# Autodesk Inventor assembly: Stadio9
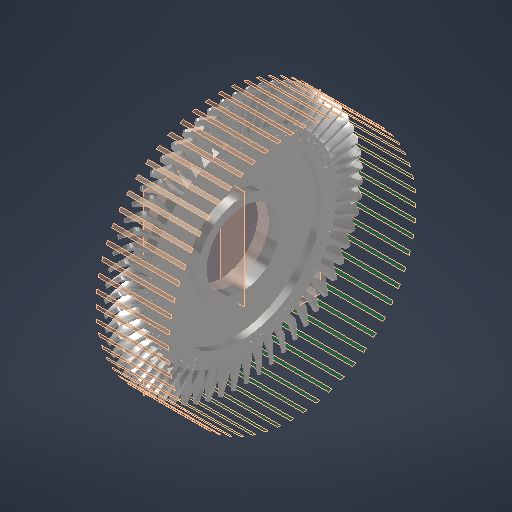
[picture p0: Inventor's stored thumbnail of the model, 512x512]
Saved by Autodesk Inventor 2026.2 (Build 302298010, 298A)
## iProperties
Created: 2026-04-25
Part Number: Stadio9
Document SubType Name: Assembly
Designer: Yan
Author: Yan
## Documents named in this file (3)
- C:\Users\Yan\Desktop\Turbina\Stadio9.iam
- C:\Users\Yan\Desktop\Turbina\DiscoPaleStadio9-DimensioniAprossimate.ipt
- C:\Users\Yan\Desktop\Turbina\PalaStadio9.ipt
## Components (61 placed, 2 different names)
1. DiscoPaleStadio9-DimensioniAprossimate:1 — Mate:1, Mate:2, Mate:3, Mate:4, Mate:5, Mate:6, Mate:7, Mate:8, Mate:9, Mate:10, Mate:11, Mate:12, Mate:13, Mate:14, Mate:15, Mate:16, Mate:17, Mate:18, Mate:19, Mate:20, Mate:21, Mate:22, Mate:23, Mate:24, Mate:25, Mate:26, Mate:27, Mate:28, Mate:30, Mate:32, Mate:33, Mate:34, Mate:35, Mate:36, Mate:37, Mate:38, Mate:39, Mate:40, Mate:41, Mate:42, Mate:43, Mate:44, Mate:45, Mate:46, Mate:47, Mate:48, Mate:49, Mate:50, Mate:51, Mate:52, Mate:53, Mate:54, Mate:55, Mate:56, Mate:57, Mate:58, Mate:59, Mate:60, Mate:61, Mate:62, Mate:63, Mate:64, Mate:65, Mate:66, Mate:67, Mate:68, Mate:69, Mate:70, Mate:71, Mate:72, Mate:73, Mate:74, Mate:75, Mate:76, Mate:77, Mate:78, Mate:79, Mate:80, Mate:81, Mate:82, Mate:83, Mate:84, Mate:85, Mate:86, Mate:87, Mate:88, Mate:89, Mate:90, Mate:91, Mate:92, Mate:93, Mate:94, Mate:95, Mate:96, Mate:97, Mate:98, Mate:99, Mate:100, Mate:101, Mate:102, Mate:103, Mate:104, Mate:105, Mate:106, Mate:107, Mate:108, Mate:109, Mate:110, Mate:111, Mate:112, Mate:113, Mate:114, Mate:115, Mate:116, Mate:117, Mate:118, Mate:119, Mate:120, Mate:121, Flush:1, Flush:2, Flush:3, Flush:4, Flush:5, Flush:6, Flush:7, Flush:8, Flush:9, Flush:10, Flush:11, Flush:12, Flush:13, Flush:14, Flush:15, Flush:16, Flush:17, Flush:18, Flush:19, Flush:20, Flush:21, Flush:22, Flush:23, Flush:24, Flush:25, Flush:26, Flush:27, Flush:28, Flush:29, Flush:30, Flush:31, Flush:32, Flush:33, Flush:34, Flush:35, Flush:36, Flush:37, Flush:38, Flush:39, Flush:40, Flush:41, Flush:42, Flush:43, Flush:44, Flush:45, Flush:46, Flush:47, Flush:48, Flush:49, Flush:50, Flush:51, Flush:52, Flush:53, Flush:54, Flush:55, Flush:56, Flush:57, Flush:58, Flush:59, Flush:60, Flush:61, Flush:62, Flush:63, Flush:64, Flush:65, Flush:66, Flush:67, Flush:68, Flush:69, Flush:70, Flush:71, Flush:72, Flush:73, Flush:74, Flush:75, Flush:76, Flush:77, Flush:78, Flush:79, Flush:80, Flush:81, Flush:82, Flush:83, Flush:84, Flush:85, Flush:86, Flush:87, Flush:88, Flush:89, Flush:90, Flush:91, Flush:92, Flush:93, Flush:94, Flush:95, Flush:96, Flush:97, Flush:98, Flush:99, Flush:100, Flush:101, Flush:102, Flush:103, Flush:104, Flush:105, Flush:106, Flush:107, Flush:108, Flush:109, Flush:110, Flush:111, Flush:112, Flush:113, Flush:114, Flush:115, Flush:116, Flush:117, Flush:118, Flush:119, Flush:120, Flush:121, Flush:122, Flush:123
2. PalaStadio9:1 — Mate:1, Mate:56, Flush:34, Flush:91
3. PalaStadio9:2 — Mate:2, Mate:55, Flush:33, Flush:90
4. PalaStadio9:3 — Mate:3, Mate:54, Flush:32, Flush:89
5. PalaStadio9:4 — Mate:4, Mate:58, Flush:31, Flush:88
6. PalaStadio9:5 — Mate:5, Mate:57, Flush:30, Flush:87
7. PalaStadio9:6 — Mate:6, Mate:53, Flush:29, Flush:86
8. PalaStadio9:7 — Mate:7, Mate:59, Flush:28, Flush:85
9. PalaStadio9:8 — Mate:8, Mate:52, Flush:27, Flush:84
10. PalaStadio9:9 — Mate:9, Mate:51, Flush:26, Flush:83
11. PalaStadio9:10 — Mate:10, Mate:50, Flush:25, Flush:82
12. PalaStadio9:11 — Mate:11, Mate:49, Flush:24, Flush:81
13. PalaStadio9:12 — Mate:12, Mate:42, Flush:23, Flush:80
14. PalaStadio9:13 — Mate:13, Mate:41, Flush:22, Flush:79
15. PalaStadio9:14 — Mate:14, Mate:48, Flush:21, Flush:78
16. PalaStadio9:15 — Mate:15, Mate:47, Flush:20, Flush:77
17. PalaStadio9:16 — Mate:16, Mate:46, Flush:19, Flush:76
18. PalaStadio9:17 — Mate:17, Mate:45, Flush:18, Flush:75
19. PalaStadio9:18 — Mate:18, Mate:40, Flush:17, Flush:74
20. PalaStadio9:19 — Mate:19, Mate:44, Flush:16, Flush:73
21. PalaStadio9:20 — Mate:20, Mate:43, Flush:15, Flush:72
22. PalaStadio9:21 — Mate:30, Mate:32, Flush:5, Flush:122
23. PalaStadio9:23 — Mate:28, Mate:60, Flush:7, Flush:61, Flush:62, Flush:64
24. PalaStadio9:24 — Mate:27, Mate:33, Flush:8, Flush:65
25. PalaStadio9:25 — Mate:26, Mate:34, Flush:9, Flush:66
26. PalaStadio9:26 — Mate:25, Mate:35, Flush:10, Flush:67
27. PalaStadio9:27 — Mate:24, Mate:36, Flush:11, Flush:68
28. PalaStadio9:28 — Mate:23, Mate:37, Flush:12, Flush:69
29. PalaStadio9:29 — Mate:22, Mate:38, Flush:13, Flush:70
30. PalaStadio9:30 — Mate:21, Mate:39, Flush:14, Flush:71
31. PalaStadio9:31 — Mate:62, Mate:65, Flush:36, Flush:93
32. PalaStadio9:32 — Mate:63, Mate:66, Flush:37, Flush:94
33. PalaStadio9:33 — Mate:67, Mate:68, Flush:38, Flush:95
34. PalaStadio9:34 — Mate:69, Mate:109, Flush:39, Flush:96
35. PalaStadio9:35 — Mate:70, Mate:110, Flush:40, Flush:97
36. PalaStadio9:36 — Mate:71, Mate:111, Flush:41, Flush:98
37. PalaStadio9:37 — Mate:72, Mate:112, Flush:42, Flush:99
38. PalaStadio9:38 — Mate:73, Mate:113, Flush:43, Flush:100
39. PalaStadio9:39 — Mate:74, Mate:114, Flush:44, Flush:101
40. PalaStadio9:40 — Mate:61, Mate:64, Flush:35, Flush:92
41. PalaStadio9:41 — Mate:75, Mate:115, Flush:45, Flush:102
42. PalaStadio9:42 — Mate:76, Mate:116, Flush:46, Flush:103
43. PalaStadio9:43 — Mate:77, Mate:117, Flush:47, Flush:104
44. PalaStadio9:44 — Mate:78, Mate:118, Flush:48, Flush:105
45. PalaStadio9:45 — Mate:79, Mate:119, Flush:49, Flush:106
46. PalaStadio9:46 — Mate:80, Flush:50, Flush:107
47. PalaStadio9:47 — Mate:81, Mate:108, Flush:51, Flush:108
48. PalaStadio9:48 — Mate:82, Mate:107, Flush:52, Flush:109
49. PalaStadio9:49 — Mate:83, Mate:106, Flush:53, Flush:110
50. PalaStadio9:50 — Mate:84, Mate:105, Flush:54, Flush:111
51. PalaStadio9:51 — Mate:85, Mate:104, Flush:55, Flush:112
52. PalaStadio9:52 — Mate:86, Mate:103, Flush:56, Flush:113
53. PalaStadio9:53 — Mate:87, Mate:102, Flush:57, Flush:114
54. PalaStadio9:54 — Mate:88, Mate:101, Flush:58, Flush:115
55. PalaStadio9:55 — Mate:89, Mate:100, Flush:59, Flush:116
56. PalaStadio9:56 — Mate:90, Mate:99, Flush:60, Flush:117
57. PalaStadio9:57 — Mate:91, Mate:98, Flush:1, Flush:118
58. PalaStadio9:58 — Mate:92, Mate:97, Flush:2, Flush:119
59. PalaStadio9:59 — Mate:93, Mate:96, Flush:3, Flush:120
60. PalaStadio9:60 — Mate:94, Mate:95, Flush:6, Flush:63, Flush:123
61. PalaStadio9:61 — Mate:120, Mate:121, Flush:4, Flush:121
## Relationships (242: Flush 123, Mate 119)
- Mate:1: DiscoPaleStadio9-DimensioniAprossimate:1 ↔ PalaStadio9:1
- Mate:2: DiscoPaleStadio9-DimensioniAprossimate:1 ↔ PalaStadio9:2
- Mate:3: DiscoPaleStadio9-DimensioniAprossimate:1 ↔ PalaStadio9:3
- Mate:4: DiscoPaleStadio9-DimensioniAprossimate:1 ↔ PalaStadio9:4
- Mate:5: DiscoPaleStadio9-DimensioniAprossimate:1 ↔ PalaStadio9:5
- Mate:6: DiscoPaleStadio9-DimensioniAprossimate:1 ↔ PalaStadio9:6
- Mate:7: DiscoPaleStadio9-DimensioniAprossimate:1 ↔ PalaStadio9:7
- Mate:8: DiscoPaleStadio9-DimensioniAprossimate:1 ↔ PalaStadio9:8
- Mate:9: DiscoPaleStadio9-DimensioniAprossimate:1 ↔ PalaStadio9:9
- Mate:10: DiscoPaleStadio9-DimensioniAprossimate:1 ↔ PalaStadio9:10
- Mate:11: DiscoPaleStadio9-DimensioniAprossimate:1 ↔ PalaStadio9:11
- Mate:12: DiscoPaleStadio9-DimensioniAprossimate:1 ↔ PalaStadio9:12
- Mate:13: DiscoPaleStadio9-DimensioniAprossimate:1 ↔ PalaStadio9:13
- Mate:14: DiscoPaleStadio9-DimensioniAprossimate:1 ↔ PalaStadio9:14
- Mate:15: DiscoPaleStadio9-DimensioniAprossimate:1 ↔ PalaStadio9:15
- Mate:16: DiscoPaleStadio9-DimensioniAprossimate:1 ↔ PalaStadio9:16
- Mate:17: DiscoPaleStadio9-DimensioniAprossimate:1 ↔ PalaStadio9:17
- Mate:18: DiscoPaleStadio9-DimensioniAprossimate:1 ↔ PalaStadio9:18
- Mate:19: DiscoPaleStadio9-DimensioniAprossimate:1 ↔ PalaStadio9:19
- Mate:20: DiscoPaleStadio9-DimensioniAprossimate:1 ↔ PalaStadio9:20
- Mate:21: DiscoPaleStadio9-DimensioniAprossimate:1 ↔ PalaStadio9:30
- Mate:22: DiscoPaleStadio9-DimensioniAprossimate:1 ↔ PalaStadio9:29
- Mate:23: DiscoPaleStadio9-DimensioniAprossimate:1 ↔ PalaStadio9:28
- Mate:24: DiscoPaleStadio9-DimensioniAprossimate:1 ↔ PalaStadio9:27
- Mate:25: DiscoPaleStadio9-DimensioniAprossimate:1 ↔ PalaStadio9:26
- Mate:26: DiscoPaleStadio9-DimensioniAprossimate:1 ↔ PalaStadio9:25
- Mate:27: DiscoPaleStadio9-DimensioniAprossimate:1 ↔ PalaStadio9:24
- Mate:28: DiscoPaleStadio9-DimensioniAprossimate:1 ↔ PalaStadio9:23
- Mate:30: DiscoPaleStadio9-DimensioniAprossimate:1 ↔ PalaStadio9:21
- Mate:32: DiscoPaleStadio9-DimensioniAprossimate:1 ↔ PalaStadio9:21
- Mate:33: DiscoPaleStadio9-DimensioniAprossimate:1 ↔ PalaStadio9:24
- Mate:34: DiscoPaleStadio9-DimensioniAprossimate:1 ↔ PalaStadio9:25
- Mate:35: DiscoPaleStadio9-DimensioniAprossimate:1 ↔ PalaStadio9:26
- Mate:36: DiscoPaleStadio9-DimensioniAprossimate:1 ↔ PalaStadio9:27
- Mate:37: DiscoPaleStadio9-DimensioniAprossimate:1 ↔ PalaStadio9:28
- Mate:38: DiscoPaleStadio9-DimensioniAprossimate:1 ↔ PalaStadio9:29
- Mate:39: DiscoPaleStadio9-DimensioniAprossimate:1 ↔ PalaStadio9:30
- Mate:40: DiscoPaleStadio9-DimensioniAprossimate:1 ↔ PalaStadio9:18
- Mate:41: DiscoPaleStadio9-DimensioniAprossimate:1 ↔ PalaStadio9:13
- Mate:42: DiscoPaleStadio9-DimensioniAprossimate:1 ↔ PalaStadio9:12
- Mate:43: DiscoPaleStadio9-DimensioniAprossimate:1 ↔ PalaStadio9:20
- Mate:44: DiscoPaleStadio9-DimensioniAprossimate:1 ↔ PalaStadio9:19
- Mate:45: DiscoPaleStadio9-DimensioniAprossimate:1 ↔ PalaStadio9:17
- Mate:46: DiscoPaleStadio9-DimensioniAprossimate:1 ↔ PalaStadio9:16
- Mate:47: DiscoPaleStadio9-DimensioniAprossimate:1 ↔ PalaStadio9:15
- Mate:48: DiscoPaleStadio9-DimensioniAprossimate:1 ↔ PalaStadio9:14
- Mate:49: DiscoPaleStadio9-DimensioniAprossimate:1 ↔ PalaStadio9:11
- Mate:50: DiscoPaleStadio9-DimensioniAprossimate:1 ↔ PalaStadio9:10
- Mate:51: DiscoPaleStadio9-DimensioniAprossimate:1 ↔ PalaStadio9:9
- Mate:52: DiscoPaleStadio9-DimensioniAprossimate:1 ↔ PalaStadio9:8
- Mate:53: DiscoPaleStadio9-DimensioniAprossimate:1 ↔ PalaStadio9:6
- Mate:54: DiscoPaleStadio9-DimensioniAprossimate:1 ↔ PalaStadio9:3
- Mate:55: DiscoPaleStadio9-DimensioniAprossimate:1 ↔ PalaStadio9:2
- Mate:56: DiscoPaleStadio9-DimensioniAprossimate:1 ↔ PalaStadio9:1
- Mate:57: DiscoPaleStadio9-DimensioniAprossimate:1 ↔ PalaStadio9:5
- Mate:58: DiscoPaleStadio9-DimensioniAprossimate:1 ↔ PalaStadio9:4
- Mate:59: DiscoPaleStadio9-DimensioniAprossimate:1 ↔ PalaStadio9:7
- Mate:60: DiscoPaleStadio9-DimensioniAprossimate:1 ↔ PalaStadio9:23
- Mate:61: DiscoPaleStadio9-DimensioniAprossimate:1 ↔ PalaStadio9:40
- Mate:62: DiscoPaleStadio9-DimensioniAprossimate:1 ↔ PalaStadio9:31
- Mate:63: DiscoPaleStadio9-DimensioniAprossimate:1 ↔ PalaStadio9:32
- Mate:64: DiscoPaleStadio9-DimensioniAprossimate:1 ↔ PalaStadio9:40
- Mate:65: DiscoPaleStadio9-DimensioniAprossimate:1 ↔ PalaStadio9:31
- Mate:66: DiscoPaleStadio9-DimensioniAprossimate:1 ↔ PalaStadio9:32
- Mate:67: DiscoPaleStadio9-DimensioniAprossimate:1 ↔ PalaStadio9:33
- Mate:68: DiscoPaleStadio9-DimensioniAprossimate:1 ↔ PalaStadio9:33
- Mate:69: DiscoPaleStadio9-DimensioniAprossimate:1 ↔ PalaStadio9:34
- Mate:70: DiscoPaleStadio9-DimensioniAprossimate:1 ↔ PalaStadio9:35
- Mate:71: DiscoPaleStadio9-DimensioniAprossimate:1 ↔ PalaStadio9:36
- Mate:72: DiscoPaleStadio9-DimensioniAprossimate:1 ↔ PalaStadio9:37
- Mate:73: DiscoPaleStadio9-DimensioniAprossimate:1 ↔ PalaStadio9:38
- Mate:74: DiscoPaleStadio9-DimensioniAprossimate:1 ↔ PalaStadio9:39
- Mate:75: DiscoPaleStadio9-DimensioniAprossimate:1 ↔ PalaStadio9:41
- Mate:76: DiscoPaleStadio9-DimensioniAprossimate:1 ↔ PalaStadio9:42
- Mate:77: DiscoPaleStadio9-DimensioniAprossimate:1 ↔ PalaStadio9:43
- Mate:78: DiscoPaleStadio9-DimensioniAprossimate:1 ↔ PalaStadio9:44
- Mate:79: DiscoPaleStadio9-DimensioniAprossimate:1 ↔ PalaStadio9:45
- Mate:80: DiscoPaleStadio9-DimensioniAprossimate:1 ↔ PalaStadio9:46
- Mate:81: DiscoPaleStadio9-DimensioniAprossimate:1 ↔ PalaStadio9:47
- Mate:82: DiscoPaleStadio9-DimensioniAprossimate:1 ↔ PalaStadio9:48
- Mate:83: DiscoPaleStadio9-DimensioniAprossimate:1 ↔ PalaStadio9:49
- Mate:84: DiscoPaleStadio9-DimensioniAprossimate:1 ↔ PalaStadio9:50
- Mate:85: DiscoPaleStadio9-DimensioniAprossimate:1 ↔ PalaStadio9:51
- Mate:86: DiscoPaleStadio9-DimensioniAprossimate:1 ↔ PalaStadio9:52
- Mate:87: DiscoPaleStadio9-DimensioniAprossimate:1 ↔ PalaStadio9:53
- Mate:88: DiscoPaleStadio9-DimensioniAprossimate:1 ↔ PalaStadio9:54
- Mate:89: DiscoPaleStadio9-DimensioniAprossimate:1 ↔ PalaStadio9:55
- Mate:90: DiscoPaleStadio9-DimensioniAprossimate:1 ↔ PalaStadio9:56
- Mate:91: DiscoPaleStadio9-DimensioniAprossimate:1 ↔ PalaStadio9:57
- Mate:92: DiscoPaleStadio9-DimensioniAprossimate:1 ↔ PalaStadio9:58
- Mate:93: DiscoPaleStadio9-DimensioniAprossimate:1 ↔ PalaStadio9:59
- Mate:94: DiscoPaleStadio9-DimensioniAprossimate:1 ↔ PalaStadio9:60
- Mate:95: DiscoPaleStadio9-DimensioniAprossimate:1 ↔ PalaStadio9:60
- Mate:96: DiscoPaleStadio9-DimensioniAprossimate:1 ↔ PalaStadio9:59
- Mate:97: DiscoPaleStadio9-DimensioniAprossimate:1 ↔ PalaStadio9:58
- Mate:98: DiscoPaleStadio9-DimensioniAprossimate:1 ↔ PalaStadio9:57
- Mate:99: DiscoPaleStadio9-DimensioniAprossimate:1 ↔ PalaStadio9:56
- Mate:100: DiscoPaleStadio9-DimensioniAprossimate:1 ↔ PalaStadio9:55
- Mate:101: DiscoPaleStadio9-DimensioniAprossimate:1 ↔ PalaStadio9:54
- Mate:102: DiscoPaleStadio9-DimensioniAprossimate:1 ↔ PalaStadio9:53
- Mate:103: DiscoPaleStadio9-DimensioniAprossimate:1 ↔ PalaStadio9:52
- Mate:104: DiscoPaleStadio9-DimensioniAprossimate:1 ↔ PalaStadio9:51
- Mate:105: DiscoPaleStadio9-DimensioniAprossimate:1 ↔ PalaStadio9:50
- Mate:106: DiscoPaleStadio9-DimensioniAprossimate:1 ↔ PalaStadio9:49
- Mate:107: DiscoPaleStadio9-DimensioniAprossimate:1 ↔ PalaStadio9:48
- Mate:108: DiscoPaleStadio9-DimensioniAprossimate:1 ↔ PalaStadio9:47
- Mate:109: DiscoPaleStadio9-DimensioniAprossimate:1 ↔ PalaStadio9:34
- Mate:110: DiscoPaleStadio9-DimensioniAprossimate:1 ↔ PalaStadio9:35
- Mate:111: DiscoPaleStadio9-DimensioniAprossimate:1 ↔ PalaStadio9:36
- Mate:112: DiscoPaleStadio9-DimensioniAprossimate:1 ↔ PalaStadio9:37
- Mate:113: DiscoPaleStadio9-DimensioniAprossimate:1 ↔ PalaStadio9:38
- Mate:114: DiscoPaleStadio9-DimensioniAprossimate:1 ↔ PalaStadio9:39
- Mate:115: DiscoPaleStadio9-DimensioniAprossimate:1 ↔ PalaStadio9:41
- Mate:116: DiscoPaleStadio9-DimensioniAprossimate:1 ↔ PalaStadio9:42
- Mate:117: DiscoPaleStadio9-DimensioniAprossimate:1 ↔ PalaStadio9:43
- Mate:118: DiscoPaleStadio9-DimensioniAprossimate:1 ↔ PalaStadio9:44
- Mate:119: DiscoPaleStadio9-DimensioniAprossimate:1 ↔ PalaStadio9:45
- Mate:120: DiscoPaleStadio9-DimensioniAprossimate:1 ↔ PalaStadio9:61
- Mate:121: DiscoPaleStadio9-DimensioniAprossimate:1 ↔ PalaStadio9:61
- Flush:1: DiscoPaleStadio9-DimensioniAprossimate:1 ↔ PalaStadio9:57
- Flush:2: DiscoPaleStadio9-DimensioniAprossimate:1 ↔ PalaStadio9:58
- Flush:3: DiscoPaleStadio9-DimensioniAprossimate:1 ↔ PalaStadio9:59
- Flush:4: DiscoPaleStadio9-DimensioniAprossimate:1 ↔ PalaStadio9:61
- Flush:5: DiscoPaleStadio9-DimensioniAprossimate:1 ↔ PalaStadio9:21
- Flush:6: DiscoPaleStadio9-DimensioniAprossimate:1 ↔ PalaStadio9:60
- Flush:7: DiscoPaleStadio9-DimensioniAprossimate:1 ↔ PalaStadio9:23
- Flush:8: DiscoPaleStadio9-DimensioniAprossimate:1 ↔ PalaStadio9:24
- Flush:9: DiscoPaleStadio9-DimensioniAprossimate:1 ↔ PalaStadio9:25
- Flush:10: DiscoPaleStadio9-DimensioniAprossimate:1 ↔ PalaStadio9:26
- Flush:11: DiscoPaleStadio9-DimensioniAprossimate:1 ↔ PalaStadio9:27
- Flush:12: DiscoPaleStadio9-DimensioniAprossimate:1 ↔ PalaStadio9:28
- Flush:13: DiscoPaleStadio9-DimensioniAprossimate:1 ↔ PalaStadio9:29
- Flush:14: DiscoPaleStadio9-DimensioniAprossimate:1 ↔ PalaStadio9:30
- Flush:15: DiscoPaleStadio9-DimensioniAprossimate:1 ↔ PalaStadio9:20
- Flush:16: DiscoPaleStadio9-DimensioniAprossimate:1 ↔ PalaStadio9:19
- Flush:17: DiscoPaleStadio9-DimensioniAprossimate:1 ↔ PalaStadio9:18
- Flush:18: DiscoPaleStadio9-DimensioniAprossimate:1 ↔ PalaStadio9:17
- Flush:19: DiscoPaleStadio9-DimensioniAprossimate:1 ↔ PalaStadio9:16
- Flush:20: DiscoPaleStadio9-DimensioniAprossimate:1 ↔ PalaStadio9:15
- Flush:21: DiscoPaleStadio9-DimensioniAprossimate:1 ↔ PalaStadio9:14
- Flush:22: DiscoPaleStadio9-DimensioniAprossimate:1 ↔ PalaStadio9:13
- Flush:23: DiscoPaleStadio9-DimensioniAprossimate:1 ↔ PalaStadio9:12
- Flush:24: DiscoPaleStadio9-DimensioniAprossimate:1 ↔ PalaStadio9:11
- Flush:25: DiscoPaleStadio9-DimensioniAprossimate:1 ↔ PalaStadio9:10
- Flush:26: DiscoPaleStadio9-DimensioniAprossimate:1 ↔ PalaStadio9:9
- Flush:27: DiscoPaleStadio9-DimensioniAprossimate:1 ↔ PalaStadio9:8
- Flush:28: DiscoPaleStadio9-DimensioniAprossimate:1 ↔ PalaStadio9:7
- Flush:29: DiscoPaleStadio9-DimensioniAprossimate:1 ↔ PalaStadio9:6
- Flush:30: DiscoPaleStadio9-DimensioniAprossimate:1 ↔ PalaStadio9:5
- Flush:31: DiscoPaleStadio9-DimensioniAprossimate:1 ↔ PalaStadio9:4
- Flush:32: DiscoPaleStadio9-DimensioniAprossimate:1 ↔ PalaStadio9:3
- Flush:33: DiscoPaleStadio9-DimensioniAprossimate:1 ↔ PalaStadio9:2
- Flush:34: DiscoPaleStadio9-DimensioniAprossimate:1 ↔ PalaStadio9:1
- Flush:35: DiscoPaleStadio9-DimensioniAprossimate:1 ↔ PalaStadio9:40
- Flush:36: DiscoPaleStadio9-DimensioniAprossimate:1 ↔ PalaStadio9:31
- Flush:37: DiscoPaleStadio9-DimensioniAprossimate:1 ↔ PalaStadio9:32
- Flush:38: DiscoPaleStadio9-DimensioniAprossimate:1 ↔ PalaStadio9:33
- Flush:39: DiscoPaleStadio9-DimensioniAprossimate:1 ↔ PalaStadio9:34
- Flush:40: DiscoPaleStadio9-DimensioniAprossimate:1 ↔ PalaStadio9:35
- Flush:41: DiscoPaleStadio9-DimensioniAprossimate:1 ↔ PalaStadio9:36
- Flush:42: DiscoPaleStadio9-DimensioniAprossimate:1 ↔ PalaStadio9:37
- Flush:43: DiscoPaleStadio9-DimensioniAprossimate:1 ↔ PalaStadio9:38
- Flush:44: DiscoPaleStadio9-DimensioniAprossimate:1 ↔ PalaStadio9:39
- Flush:45: DiscoPaleStadio9-DimensioniAprossimate:1 ↔ PalaStadio9:41
- Flush:46: DiscoPaleStadio9-DimensioniAprossimate:1 ↔ PalaStadio9:42
- Flush:47: DiscoPaleStadio9-DimensioniAprossimate:1 ↔ PalaStadio9:43
- Flush:48: DiscoPaleStadio9-DimensioniAprossimate:1 ↔ PalaStadio9:44
- Flush:49: DiscoPaleStadio9-DimensioniAprossimate:1 ↔ PalaStadio9:45
- Flush:50: DiscoPaleStadio9-DimensioniAprossimate:1 ↔ PalaStadio9:46
- Flush:51: DiscoPaleStadio9-DimensioniAprossimate:1 ↔ PalaStadio9:47
- Flush:52: DiscoPaleStadio9-DimensioniAprossimate:1 ↔ PalaStadio9:48
- Flush:53: DiscoPaleStadio9-DimensioniAprossimate:1 ↔ PalaStadio9:49
- Flush:54: DiscoPaleStadio9-DimensioniAprossimate:1 ↔ PalaStadio9:50
- Flush:55: DiscoPaleStadio9-DimensioniAprossimate:1 ↔ PalaStadio9:51
- Flush:56: DiscoPaleStadio9-DimensioniAprossimate:1 ↔ PalaStadio9:52
- Flush:57: DiscoPaleStadio9-DimensioniAprossimate:1 ↔ PalaStadio9:53
- Flush:58: DiscoPaleStadio9-DimensioniAprossimate:1 ↔ PalaStadio9:54
- Flush:59: DiscoPaleStadio9-DimensioniAprossimate:1 ↔ PalaStadio9:55
- Flush:60: DiscoPaleStadio9-DimensioniAprossimate:1 ↔ PalaStadio9:56
- Flush:61: DiscoPaleStadio9-DimensioniAprossimate:1 ↔ PalaStadio9:23
- Flush:62: DiscoPaleStadio9-DimensioniAprossimate:1 ↔ PalaStadio9:23
- Flush:63: DiscoPaleStadio9-DimensioniAprossimate:1 ↔ PalaStadio9:60
- Flush:64: DiscoPaleStadio9-DimensioniAprossimate:1 ↔ PalaStadio9:23
- Flush:65: DiscoPaleStadio9-DimensioniAprossimate:1 ↔ PalaStadio9:24
- Flush:66: DiscoPaleStadio9-DimensioniAprossimate:1 ↔ PalaStadio9:25
- Flush:67: DiscoPaleStadio9-DimensioniAprossimate:1 ↔ PalaStadio9:26
- Flush:68: DiscoPaleStadio9-DimensioniAprossimate:1 ↔ PalaStadio9:27
- Flush:69: DiscoPaleStadio9-DimensioniAprossimate:1 ↔ PalaStadio9:28
- Flush:70: DiscoPaleStadio9-DimensioniAprossimate:1 ↔ PalaStadio9:29
- Flush:71: DiscoPaleStadio9-DimensioniAprossimate:1 ↔ PalaStadio9:30
- Flush:72: DiscoPaleStadio9-DimensioniAprossimate:1 ↔ PalaStadio9:20
- Flush:73: DiscoPaleStadio9-DimensioniAprossimate:1 ↔ PalaStadio9:19
- Flush:74: DiscoPaleStadio9-DimensioniAprossimate:1 ↔ PalaStadio9:18
- Flush:75: DiscoPaleStadio9-DimensioniAprossimate:1 ↔ PalaStadio9:17
- Flush:76: DiscoPaleStadio9-DimensioniAprossimate:1 ↔ PalaStadio9:16
- Flush:77: DiscoPaleStadio9-DimensioniAprossimate:1 ↔ PalaStadio9:15
- Flush:78: DiscoPaleStadio9-DimensioniAprossimate:1 ↔ PalaStadio9:14
- Flush:79: DiscoPaleStadio9-DimensioniAprossimate:1 ↔ PalaStadio9:13
- Flush:80: DiscoPaleStadio9-DimensioniAprossimate:1 ↔ PalaStadio9:12
- Flush:81: DiscoPaleStadio9-DimensioniAprossimate:1 ↔ PalaStadio9:11
- Flush:82: DiscoPaleStadio9-DimensioniAprossimate:1 ↔ PalaStadio9:10
- Flush:83: DiscoPaleStadio9-DimensioniAprossimate:1 ↔ PalaStadio9:9
- Flush:84: DiscoPaleStadio9-DimensioniAprossimate:1 ↔ PalaStadio9:8
- Flush:85: DiscoPaleStadio9-DimensioniAprossimate:1 ↔ PalaStadio9:7
- Flush:86: DiscoPaleStadio9-DimensioniAprossimate:1 ↔ PalaStadio9:6
- Flush:87: DiscoPaleStadio9-DimensioniAprossimate:1 ↔ PalaStadio9:5
- Flush:88: DiscoPaleStadio9-DimensioniAprossimate:1 ↔ PalaStadio9:4
- Flush:89: DiscoPaleStadio9-DimensioniAprossimate:1 ↔ PalaStadio9:3
- Flush:90: DiscoPaleStadio9-DimensioniAprossimate:1 ↔ PalaStadio9:2
- Flush:91: DiscoPaleStadio9-DimensioniAprossimate:1 ↔ PalaStadio9:1
- Flush:92: DiscoPaleStadio9-DimensioniAprossimate:1 ↔ PalaStadio9:40
- Flush:93: DiscoPaleStadio9-DimensioniAprossimate:1 ↔ PalaStadio9:31
- Flush:94: DiscoPaleStadio9-DimensioniAprossimate:1 ↔ PalaStadio9:32
- Flush:95: DiscoPaleStadio9-DimensioniAprossimate:1 ↔ PalaStadio9:33
- Flush:96: DiscoPaleStadio9-DimensioniAprossimate:1 ↔ PalaStadio9:34
- Flush:97: DiscoPaleStadio9-DimensioniAprossimate:1 ↔ PalaStadio9:35
- Flush:98: DiscoPaleStadio9-DimensioniAprossimate:1 ↔ PalaStadio9:36
- Flush:99: DiscoPaleStadio9-DimensioniAprossimate:1 ↔ PalaStadio9:37
- Flush:100: DiscoPaleStadio9-DimensioniAprossimate:1 ↔ PalaStadio9:38
- Flush:101: DiscoPaleStadio9-DimensioniAprossimate:1 ↔ PalaStadio9:39
- Flush:102: DiscoPaleStadio9-DimensioniAprossimate:1 ↔ PalaStadio9:41
- Flush:103: DiscoPaleStadio9-DimensioniAprossimate:1 ↔ PalaStadio9:42
- Flush:104: DiscoPaleStadio9-DimensioniAprossimate:1 ↔ PalaStadio9:43
- Flush:105: DiscoPaleStadio9-DimensioniAprossimate:1 ↔ PalaStadio9:44
- Flush:106: DiscoPaleStadio9-DimensioniAprossimate:1 ↔ PalaStadio9:45
- Flush:107: DiscoPaleStadio9-DimensioniAprossimate:1 ↔ PalaStadio9:46
- Flush:108: DiscoPaleStadio9-DimensioniAprossimate:1 ↔ PalaStadio9:47
- Flush:109: DiscoPaleStadio9-DimensioniAprossimate:1 ↔ PalaStadio9:48
- Flush:110: DiscoPaleStadio9-DimensioniAprossimate:1 ↔ PalaStadio9:49
- Flush:111: DiscoPaleStadio9-DimensioniAprossimate:1 ↔ PalaStadio9:50
- Flush:112: DiscoPaleStadio9-DimensioniAprossimate:1 ↔ PalaStadio9:51
- Flush:113: DiscoPaleStadio9-DimensioniAprossimate:1 ↔ PalaStadio9:52
- Flush:114: DiscoPaleStadio9-DimensioniAprossimate:1 ↔ PalaStadio9:53
- Flush:115: DiscoPaleStadio9-DimensioniAprossimate:1 ↔ PalaStadio9:54
- Flush:116: DiscoPaleStadio9-DimensioniAprossimate:1 ↔ PalaStadio9:55
- Flush:117: DiscoPaleStadio9-DimensioniAprossimate:1 ↔ PalaStadio9:56
- Flush:118: DiscoPaleStadio9-DimensioniAprossimate:1 ↔ PalaStadio9:57
- Flush:119: DiscoPaleStadio9-DimensioniAprossimate:1 ↔ PalaStadio9:58
- Flush:120: DiscoPaleStadio9-DimensioniAprossimate:1 ↔ PalaStadio9:59
- Flush:121: DiscoPaleStadio9-DimensioniAprossimate:1 ↔ PalaStadio9:61
- Flush:122: DiscoPaleStadio9-DimensioniAprossimate:1 ↔ PalaStadio9:21
- Flush:123: DiscoPaleStadio9-DimensioniAprossimate:1 ↔ PalaStadio9:60
